# Autodesk Inventor assembly: RaspiPly
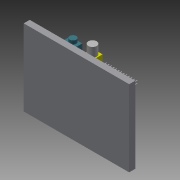
[picture p0: Inventor's stored thumbnail of the model, 180x180]
Saved by Autodesk Inventor 2015 (Build 190159000, 159)
## iProperties
Created: 2014-04-26
Part Number: RaspiPly
Document SubType Name: Assembly
Designer: Jack
Author: Jack
## Documents named in this file (3)
- C:\Users\Jack\Sync\MendelMax1.5\InventorParts\Electronics\RaspiPly.iam
- C:\Users\Jack\Sync\MendelMax1.5\InventorParts\Electronics\Raspi.ipt
- C:\Users\Jack\Sync\MendelMax1.5\InventorParts\Electronics\RaspiPly.ipt
## Components (2 placed, 2 different names)
1. Raspi:1 — Mate:1, Flush:1, Flush:2
2. RaspiPly:1 — Mate:1, Flush:1, Flush:2
## Relationships (3: Flush 2, Mate 1)
- Mate:1: Raspi:1 ↔ RaspiPly:1
- Flush:1 (-10 mm): Raspi:1 ↔ RaspiPly:1
- Flush:2 (-10 mm): Raspi:1 ↔ RaspiPly:1
